# Autodesk Inventor assembly: Transmisión por cadena
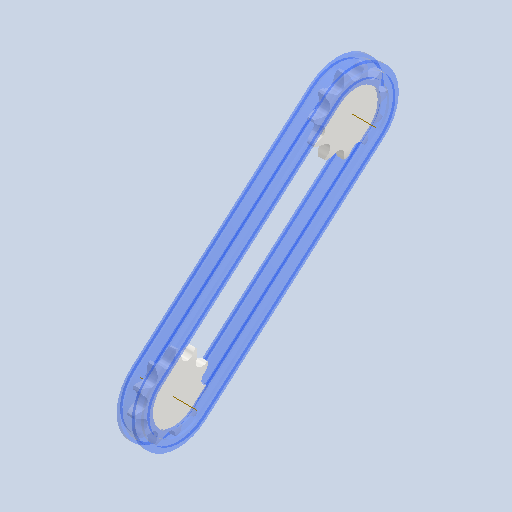
[picture p0: Inventor's stored thumbnail of the model, 512x512]
Saved by Autodesk Inventor 2022.1 (Build 261234000, 234)
## iProperties
ClientObjectVersion: 1
Created: 2021-09-12
Part Number: Transmisión por cadena
Document SubType Name: Assembly
Designer: seb_0
Author: seb_0
## Documents named in this file (4)
- C:\Users\seb_0\Desktop\RobotPallet_v2\Mecanismo de movimiento\Mecanismo - Derecho\Design Accelerator\Transmisión por cadena1.iam
- C:\Users\seb_0\Desktop\RobotPallet_v2\Mecanismo de movimiento\Mecanismo - Derecho\Design Accelerator\Cadena de rodillos1.ipt
- C:\Users\seb_0\Desktop\RobotPallet_v2\Mecanismo de movimiento\Mecanismo - Derecho\Design Accelerator\Rueda dentada de cadena de rodillos11.ipt
- C:\Users\seb_0\Desktop\RobotPallet_v2\Mecanismo de movimiento\Mecanismo - Derecho\Design Accelerator\Rueda dentada de cadena de rodillos21.ipt
## Components (3 placed, 3 different names)
1. Cadena de rodillos:1 — Nivelación:1, Coincidencia:1, Coincidencia:2, Nivelación:2, Coincidencia:3, Coincidencia:4
2. Rueda dentada de cadena de rodillos1:1 — Nivelación:1, Coincidencia:1, Coincidencia:2, Rotación:1
3. Rueda dentada de cadena de rodillos2:1 — Nivelación:2, Coincidencia:3, Rotación:1, Coincidencia:4
## Relationships (7: Mate 4, Flush 2, RelateRotation 1)
- Nivelación:1 [Flush]: Cadena de rodillos:1 ↔ Rueda dentada de cadena de rodillos1:1
- Coincidencia:1 [Mate]: Cadena de rodillos:1 ↔ Rueda dentada de cadena de rodillos1:1
- Coincidencia:2 [Mate]: Cadena de rodillos:1 ↔ Rueda dentada de cadena de rodillos1:1
- Nivelación:2 [Flush]: Cadena de rodillos:1 ↔ Rueda dentada de cadena de rodillos2:1
- Coincidencia:3 [Mate]: Cadena de rodillos:1 ↔ Rueda dentada de cadena de rodillos2:1
- Rotación:1 [RelateRotation] (1 ul): Rueda dentada de cadena de rodillos1:1 ↔ Rueda dentada de cadena de rodillos2:1
- Coincidencia:4 [Mate]: Cadena de rodillos:1 ↔ Rueda dentada de cadena de rodillos2:1
